# Autodesk Inventor assembly: LCD
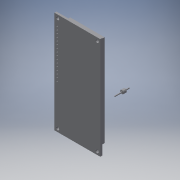
[picture p0: Inventor's stored thumbnail of the model, 180x180]
Saved by Autodesk Inventor 2016 (Build 200138000, 138)
## iProperties
Created: 2016-04-16
Part Number: LCD
Document SubType Name: Assembly
Designer: Jarrett
Author: Jarrett
## Documents named in this file (5)
- C:\Users\Jarrett\Dropbox (Personal)\Ergo Systems\Projects\yarndyer\CAD\LCD\LCD.iam
- C:\Users\Jarrett\Dropbox (Personal)\Ergo Systems\Projects\yarndyer\CAD\LCD\PCB.ipt
- C:\Users\Jarrett\Dropbox (Personal)\Ergo Systems\Projects\yarndyer\CAD\LCD\LCD Module.ipt
- C:\Users\Jarrett\Dropbox (Personal)\Ergo Systems\Projects\yarndyer\CAD\LCD\Pin Shroud.ipt
- C:\Users\Jarrett\Dropbox (Personal)\Ergo Systems\Projects\yarndyer\CAD\LCD\Pin.ipt
## Components (4 placed, 4 different names)
1. PCB:1 — Mate:1, Flush:1, Flush:2
2. LCD Module:1 — Mate:1, Flush:1, Flush:2
3. Pin Shroud:1 — Mate:4, Mate:2, Flush:3
4. Pin:1 — Mate:4, Mate:2, Flush:3
## Relationships (6: Mate 3, Flush 3)
- Mate:1: PCB:1 ↔ LCD Module:1
- Flush:1 (4.6 mm): PCB:1 ↔ LCD Module:1
- Flush:2 (4.2 mm): PCB:1 ↔ LCD Module:1
- Mate:4: Pin Shroud:1 ↔ Pin:1
- Mate:2: Pin Shroud:1 ↔ Pin:1
- Flush:3 (3.5 mm): Pin Shroud:1 ↔ Pin:1
